# Autodesk Inventor assembly: beep_rgb_ir_assembled_2
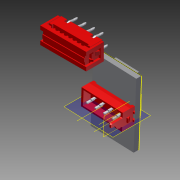
[picture p0: Inventor's stored thumbnail of the model, 180x180]
Saved by Autodesk Inventor 2014 (Build 180170000, 170)
## iProperties
Created: 2013-08-25
Part Number: beep_rgb_ir_assembled_2
Document SubType Name: Assembly
Designer: Felix
Author: Felix
## Documents named in this file (6)
- C:\Users\Felix\Desktop\Beep\Hardware\3D-CAD\parts\electronic\BEEP\beep_rgb_ir_assembled_2.iam
- C:\Users\Felix\Desktop\Beep\Hardware\3D-CAD\parts\electronic\BEEP\beep_rgb_ir.ipt
- C:\Users\Felix\Desktop\Beep\Hardware\3D-CAD\parts\electronic\BEEP\components\HSDL-9100-024\HSDL-9100.iam
- C:\Users\Felix\Desktop\Beep\Hardware\3D-CAD\parts\electronic\BEEP\components\micro-miniature_steckverbinder_a-30-08p-1300.ipt
- C:\Users\Felix\Desktop\Beep\Hardware\3D-CAD\parts\electronic\BEEP\components\5050 LED\5050_LED.ipt
- C:\Users\Felix\Desktop\Beep\Hardware\3D-CAD\parts\electronic\BEEP\components\micro-miniature_steckverbinder_a-31-08p-1300.iam
## Components (5 placed, 5 different names)
1. beep_rgb_ir:1 — Passend:5, Passend:9, Passend:10, Passend:11, Passend:12, Passend:13, Passend:14, Passend:15, Passend:16, Passend:17, Passend:18
2. HSDL-9100:1 [sub-assembly] — Passend:5, Passend:16, Passend:17
3. micro-miniature_steckverbinder_a-30-08p-1300:1 — Passend:9, Passend:10, Passend:11, Passend:12
4. 5050_LED:1 — Passend:13, Passend:14, Passend:15
5. micro-miniature_steckverbinder_a-31-08p-1300:1 [sub-assembly] — Passend:18
## Relationships (11: Mate 11)
- Passend:5 [Mate]: beep_rgb_ir:1 ↔ HSDL-9100:1
- Passend:9 [Mate]: beep_rgb_ir:1 ↔ micro-miniature_steckverbinder_a-30-08p-1300:1
- Passend:10 [Mate]: beep_rgb_ir:1 ↔ micro-miniature_steckverbinder_a-30-08p-1300:1
- Passend:11 [Mate]: beep_rgb_ir:1 ↔ micro-miniature_steckverbinder_a-30-08p-1300:1
- Passend:12 [Mate]: beep_rgb_ir:1 ↔ micro-miniature_steckverbinder_a-30-08p-1300:1
- Passend:13 [Mate]: beep_rgb_ir:1 ↔ 5050_LED:1
- Passend:14 [Mate]: beep_rgb_ir:1 ↔ 5050_LED:1
- Passend:15 [Mate]: beep_rgb_ir:1 ↔ 5050_LED:1
- Passend:16 [Mate]: beep_rgb_ir:1 ↔ HSDL-9100:1
- Passend:17 [Mate]: beep_rgb_ir:1 ↔ HSDL-9100:1
- Passend:18 [Mate]: beep_rgb_ir:1 ↔ micro-miniature_steckverbinder_a-31-08p-1300:1
